# Autodesk Inventor assembly: 三号螺丝+螺帽套
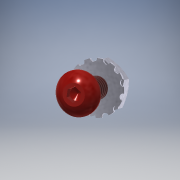
[picture p0: Inventor's stored thumbnail of the model, 180x180]
Saved by Autodesk Inventor 2019.4 (Build 234330000, 330)
## iProperties
Created: 2018-09-03
Part Number: 三号螺丝+螺帽套
Material: 常规
Document SubType Name: Assembly
Designer: aresp
Mass: 3.28505 g
Surface Area: 6.70102 cm^2
Volume: 0.424519 cm^3
Density: 7.7383 g/cm^3
d2: 0.000 mm
d1_d2: 0.000 mm
Author: aresp
## Documents named in this file (3)
- D:\towerTakeOverCad\ncrCadLib\三号螺丝+螺帽套.iam
- D:\towerTakeOverCad\ncrCadLib\螺丝螺帽\Screw 8-32 x 0.500'' - Black.ipt
- D:\towerTakeOverCad\ncrCadLib\螺丝螺帽\Nut 8-32 Keps.ipt
## Components (2 placed, 2 different names)
1. Screw 8-32 x 0.500'' - Black:1
2. Nut 8-32 Keps:1
## Named parameters: d1_d2 = 0 mm
